# Autodesk Inventor assembly: Ladder Mech
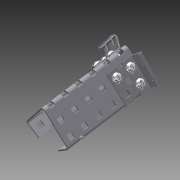
[picture p0: Inventor's stored thumbnail of the model, 180x180]
Saved by Autodesk Inventor 2012 (Build 160160000, 160)
## iProperties
Created: 2011-09-20
Part Number: Ladder Mech
Document SubType Name: Assembly
Designer: Wade
Author: Wade
## Documents named in this file (4)
- C:\Users\Wade\Documents\1103 Robot - CAD Assembly\Ladder Mech.iam
- C:\Users\Wade\Documents\1103 Robot - CAD Assembly\Custom Bent C Channel (ladder).ipt
- C:\Users\Wade\Documents\1103 Robot - CAD Assembly\Ladder Hook.ipt
- C:\Users\Wade\Documents\1103 Robot - CAD Assembly\.375'' Screw & Nylock Nut.iam
## Components (9 placed, 3 different names)
1. Custom Bent C Channel (ladder):1 — Mate:1, Mate:2, Flush:1, Flush:2, Flush:3, Mate:3, Mate:8, Mate:11
2. Ladder Hook:1 — Mate:1, Flush:3, Mate:3, Mate:13, Mate:14, Mate:15, Mate:16, Mate:17, Mate:18, Mate:19, Mate:20, Mate:21
3. Ladder Hook:2 — Mate:2, Flush:1, Flush:2, Mate:4, Mate:5, Mate:6, Mate:7, Mate:9, Mate:10, Mate:12
4. .375'' Screw & Nylock Nut:1 [sub-assembly] — Mate:7, Mate:8, Mate:9
5. .375'' Screw & Nylock Nut:2 [sub-assembly] — Mate:4, Mate:5, Mate:6
6. .375'' Screw & Nylock Nut:3 [sub-assembly] — Mate:10, Mate:11, Mate:12
7. .375'' Screw & Nylock Nut:4 [sub-assembly] — Mate:13, Mate:14, Mate:15
8. .375'' Screw & Nylock Nut:5 [sub-assembly] — Mate:19, Mate:20, Mate:21
9. .375'' Screw & Nylock Nut:6 [sub-assembly] — Mate:16, Mate:17, Mate:18
## Relationships (24: Mate 21, Flush 3)
- Mate:1: Custom Bent C Channel (ladder):1 ↔ Ladder Hook:1
- Mate:2: Custom Bent C Channel (ladder):1 ↔ Ladder Hook:2
- Flush:1: Custom Bent C Channel (ladder):1 ↔ Ladder Hook:2
- Flush:2: Custom Bent C Channel (ladder):1 ↔ Ladder Hook:2
- Flush:3: Custom Bent C Channel (ladder):1 ↔ Ladder Hook:1
- Mate:3: Custom Bent C Channel (ladder):1 ↔ Ladder Hook:1
- Mate:4 (2.3114 mm): Ladder Hook:2 ↔ .375'' Screw & Nylock Nut:2
- Mate:5 (2.3114 mm): Ladder Hook:2 ↔ .375'' Screw & Nylock Nut:2
- Mate:6: Ladder Hook:2 ↔ .375'' Screw & Nylock Nut:2
- Mate:7 (2.3114 mm): Ladder Hook:2 ↔ .375'' Screw & Nylock Nut:1
- Mate:8 (2.3114 mm): Custom Bent C Channel (ladder):1 ↔ .375'' Screw & Nylock Nut:1
- Mate:9: Ladder Hook:2 ↔ .375'' Screw & Nylock Nut:1
- Mate:10 (2.3114 mm): Ladder Hook:2 ↔ .375'' Screw & Nylock Nut:3
- Mate:11 (2.3114 mm): Custom Bent C Channel (ladder):1 ↔ .375'' Screw & Nylock Nut:3
- Mate:12: Ladder Hook:2 ↔ .375'' Screw & Nylock Nut:3
- Mate:13 (2.3114 mm): Ladder Hook:1 ↔ .375'' Screw & Nylock Nut:4
- Mate:14 (2.3114 mm): Ladder Hook:1 ↔ .375'' Screw & Nylock Nut:4
- Mate:15: Ladder Hook:1 ↔ .375'' Screw & Nylock Nut:4
- Mate:16 (2.3114 mm): Ladder Hook:1 ↔ .375'' Screw & Nylock Nut:6
- Mate:17 (2.3114 mm): Ladder Hook:1 ↔ .375'' Screw & Nylock Nut:6
- Mate:18: Ladder Hook:1 ↔ .375'' Screw & Nylock Nut:6
- Mate:19 (2.3114 mm): Ladder Hook:1 ↔ .375'' Screw & Nylock Nut:5
- Mate:20 (2.3114 mm): Ladder Hook:1 ↔ .375'' Screw & Nylock Nut:5
- Mate:21: Ladder Hook:1 ↔ .375'' Screw & Nylock Nut:5
